# Autodesk Inventor assembly: Rov1
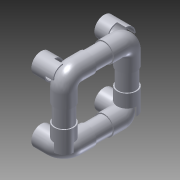
[picture p0: Inventor's stored thumbnail of the model, 180x180]
Saved by Autodesk Inventor 2013 (Build 170138000, 138)
## iProperties
Created: 2013-06-24
Part Number: Rov1
Document SubType Name: Assembly
Designer: Kyle
Author: Kyle
## Documents named in this file (3)
- C:\Users\Kyle\Documents\Inventor\2013\ROV\Rov1.iam
- C:\Users\Kyle\Documents\Inventor\2013\ROV\3 Way Corner.ipt
- C:\Users\Kyle\Documents\Inventor\2013\ROV\2.5 pipe.ipt
## Components (8 placed, 2 different names)
1. 3 Way Corner:1 — Mate:1, Mate:2, Flush:1, Mate:7, Mate:8, Flush:2
2. 3 Way Corner:2 — Mate:3, Flush:1, Mate:4, Mate:5, Mate:6
3. 2.5 pipe:1 — Mate:1, Mate:2, Mate:3, Mate:4
4. 3 Way Corner:3 — Mate:10, Mate:11, Flush:2, Mate:12, Mate:13
5. 3 Way Corner:4 — Mate:14, Mate:15, Mate:16, Mate:17
6. 2.5 pipe:2 — Mate:12, Mate:13, Mate:14, Mate:16
7. 2.5 pipe:3 — Mate:5, Mate:6, Mate:15, Mate:17
8. 2.5 pipe:4 — Mate:7, Mate:8, Mate:10, Mate:11
## Relationships (18: Mate 16, Flush 2)
- Mate:1: 3 Way Corner:1 ↔ 2.5 pipe:1
- Mate:2 (-19.05 mm): 3 Way Corner:1 ↔ 2.5 pipe:1
- Mate:3 (-19.05 mm): 3 Way Corner:2 ↔ 2.5 pipe:1
- Flush:1: 3 Way Corner:1 ↔ 3 Way Corner:2
- Mate:4: 3 Way Corner:2 ↔ 2.5 pipe:1
- Mate:5: 3 Way Corner:2 ↔ 2.5 pipe:3
- Mate:6 (-19.05 mm): 3 Way Corner:2 ↔ 2.5 pipe:3
- Mate:7: 3 Way Corner:1 ↔ 2.5 pipe:4
- Mate:8 (-19.05 mm): 3 Way Corner:1 ↔ 2.5 pipe:4
- Mate:10: 3 Way Corner:3 ↔ 2.5 pipe:4
- Mate:11 (-19.05 mm): 3 Way Corner:3 ↔ 2.5 pipe:4
- Flush:2: 3 Way Corner:1 ↔ 3 Way Corner:3
- Mate:12: 3 Way Corner:3 ↔ 2.5 pipe:2
- Mate:13 (-19.05 mm): 3 Way Corner:3 ↔ 2.5 pipe:2
- Mate:14 (-19.05 mm): 3 Way Corner:4 ↔ 2.5 pipe:2
- Mate:15 (-19.05 mm): 3 Way Corner:4 ↔ 2.5 pipe:3
- Mate:16: 3 Way Corner:4 ↔ 2.5 pipe:2
- Mate:17: 3 Way Corner:4 ↔ 2.5 pipe:3
